# Autodesk Inventor assembly: coxa kiri
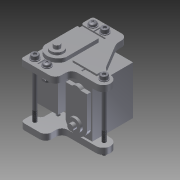
[picture p0: Inventor's stored thumbnail of the model, 180x180]
Saved by Autodesk Inventor 2012 (Build 160160000, 160)
## iProperties
Created: 2013-12-07
Part Number: coxa kiri
Document SubType Name: Assembly
Designer: Irwan Haryanto
Author: Irwan Haryanto
## Documents named in this file (9)
- D:\Revenant\robot baru 2014\coxa kiri.iam
- D:\Revenant\robot baru 2014\braket atas.ipt
- D:\Revenant\robot baru 2014\braket bawah.ipt
- D:\Revenant\robot baru 2014\servo HS-7955GT.ipt
- D:\Revenant\robot baru 2014\coxa kiri\Design Accelerator\Bolted Connection1.iam
- D:\Revenant\robot baru 2014\coxa kiri\Design Accelerator\Bolted Connection2.iam
- D:\Revenant\robot baru 2014\coxa kiri\Design Accelerator\Bolted Connection3.iam
- D:\Revenant\robot baru 2014\coxa kiri\Design Accelerator\Bolted Connection4.iam
- D:\Revenant\robot baru 2014\coxa kiri\Design Accelerator\Bolted Connection5.iam
## Components (9 placed, 4 different names)
1. braket atas:1 — Mate:1, Mate:2, Mate:3, Insert:1, Insert:2, Mate:7, Mate:9, Mate:11, Mate:13, Mate:15
2. servo HS-7955GT:1 — Mate:1, Mate:2, Mate:3, Mate:4, Mate:5, Mate:6
3. servo HS-7955GT:2 — Insert:1, Insert:2, Mate:14, Mate:16
4. braket bawah:1 — Mate:4, Mate:5, Mate:6, Mate:8, Mate:10, Mate:12
5. Bolted Connection:1 [sub-assembly] — Mate:7, Mate:8
6. Bolted Connection:2 [sub-assembly] — Mate:9, Mate:10
7. Bolted Connection:3 [sub-assembly] — Mate:11, Mate:12
8. Bolted Connection:4 [sub-assembly] — Mate:13, Mate:14
9. Bolted Connection:5 [sub-assembly] — Mate:15, Mate:16
## Relationships (18: Mate 16, Insert 2)
- Mate:1: braket atas:1 ↔ servo HS-7955GT:1
- Mate:2: braket atas:1 ↔ servo HS-7955GT:1
- Mate:3: braket atas:1 ↔ servo HS-7955GT:1
- Mate:4: servo HS-7955GT:1 ↔ braket bawah:1
- Mate:5: servo HS-7955GT:1 ↔ braket bawah:1
- Mate:6: servo HS-7955GT:1 ↔ braket bawah:1
- Insert:1: braket atas:1 ↔ servo HS-7955GT:2
- Insert:2: braket atas:1 ↔ servo HS-7955GT:2
- Mate:7: braket atas:1 ↔ Bolted Connection:1
- Mate:8: braket bawah:1 ↔ Bolted Connection:1
- Mate:9: braket atas:1 ↔ Bolted Connection:2
- Mate:10: braket bawah:1 ↔ Bolted Connection:2
- Mate:11: braket atas:1 ↔ Bolted Connection:3
- Mate:12: braket bawah:1 ↔ Bolted Connection:3
- Mate:13: braket atas:1 ↔ Bolted Connection:4
- Mate:14: servo HS-7955GT:2 ↔ Bolted Connection:4
- Mate:15: braket atas:1 ↔ Bolted Connection:5
- Mate:16: servo HS-7955GT:2 ↔ Bolted Connection:5
